# Autodesk Inventor assembly: k400+ полная
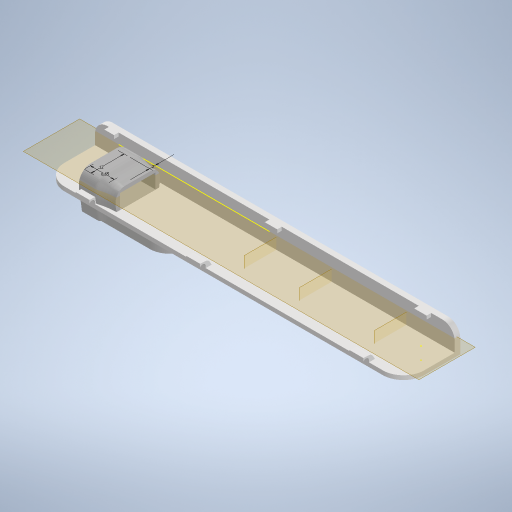
[picture p0: Inventor's stored thumbnail of the model, 512x512]
Saved by Autodesk Inventor 2024.2 (Build 282272000, 272)
## iProperties
Created: 2025-12-06
Part Number: k400+ полная
Document SubType Name: Assembly
Designer: Zakhar
Author: Zakhar
## Documents named in this file (3)
- C:\Users\Zakhar\Documents\Artist\3D\стл\k400+ полная.iam
- C:\Users\Zakhar\Documents\Artist\3D\стл\k400+ крышка.ipt
- F:\downloads\Telegram Desktop\JBL USB Holder-v2.ipt
## Components (2 placed, 2 different names)
1. k400+ крышка:1 — Совмещение:2, Совмещение:3
2. JBL USB Holder-v2:1 — Совмещение:2, Совмещение:3
## Relationships (2: Mate 2)
- Совмещение:2 [Mate] (-5.8 mm): k400+ крышка:1 ↔ JBL USB Holder-v2:1
- Совмещение:3 [Mate] (2 mm): k400+ крышка:1 ↔ JBL USB Holder-v2:1
